# Autodesk Inventor assembly: BracketAssembly
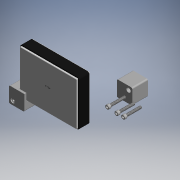
[picture p0: Inventor's stored thumbnail of the model, 180x180]
Saved by Autodesk Inventor 2016 (Build 200138000, 138)
## iProperties
Created: 2015-10-05
Part Number: BracketAssembly
Document SubType Name: Assembly
Designer: steele
Author: steele
## Documents named in this file (4)
- C:\snobotics\CAD-Development\robSteele\SnoBoticsSummer2015\BracketForDLink\BracketAssembly.iam
- C:\snobotics\autodesk\2015\FRC_KOP_2015\Control System\CS_WirelessBridge_DAP1522.ipt
- C:\snobotics\CAD-Development\robSteele\SnoBoticsSummer2015\BracketForDLink\cornerBracketForDLink.ipt
- C:\snobotics\CAD-MfgResources\McMaster-Carr\Cap Screws\Black-Oxide Alloy Steel\1_4_20x1_5_in_long\90044A123.ipt
## Components (7 placed, 3 different names)
1. CS_WirelessBridge_DAP1522:1 — Mate:1, Mate:2, Flush:1
2. cornerBracketForDLink:1 — Mate:1, Mate:2, Flush:1, Insert:1
3. cornerBracketForDLink:2
4. 90044A123:1 — Insert:1
5. 90044A123:2
6. 90044A123:3
7. 90044A123:4
## Relationships (4: Mate 2, Flush 1, Insert 1)
- Mate:1: CS_WirelessBridge_DAP1522:1 ↔ cornerBracketForDLink:1
- Mate:2: CS_WirelessBridge_DAP1522:1 ↔ cornerBracketForDLink:1
- Flush:1: CS_WirelessBridge_DAP1522:1 ↔ cornerBracketForDLink:1
- Insert:1: cornerBracketForDLink:1 ↔ 90044A123:1
